# Autodesk Inventor assembly: Tower Pro 9g Micro Servo SG90
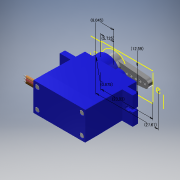
[picture p0: Inventor's stored thumbnail of the model, 180x180]
Saved by Autodesk Inventor 2017 (Build 210142000, 142)
## iProperties
Created: 2015-05-27
Part Number: Tower Pro 9g Micro Servo SG90
Material: 一般
Document SubType Name: Assembly
Designer: sktom
Sending System: SolidWorks 2014
Last Author: Simon
Last Saved: 2015-06-03
Author: sktom
## Documents named in this file (3)
- D:\OneDrive\CAD\MAJ\hackberry\HACKberry-hardware\3D_69%inlength\Inventor\HbHandForChild\servo\Tower Pro 9g Micro Servo SG90.iam
- D:\OneDrive\CAD\MAJ\hackberry\HACKberry-hardware\3D_69%inlength\Inventor\HbHandForChild\servo\Tower Pro 9g Micro Servo SG90.ipt
- D:\OneDrive\CAD\MAJ\hackberry\HACKberry-hardware\3D_69%inlength\Inventor\HbHandForChild\servo\SG90 plastic Horn.ipt
## Components (2 placed, 2 different names)
1. Tower Pro 9g Micro Servo SG90:1 — 挿入:1
2. SG90 plastic Horn:1 — 挿入:1
## Relationships (1: Insert 1)
- 挿入:1 [Insert]: Tower Pro 9g Micro Servo SG90:1 ↔ SG90 plastic Horn:1
